# Autodesk Inventor assembly: pince
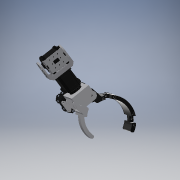
[picture p0: Inventor's stored thumbnail of the model, 180x180]
Saved by Autodesk Inventor 2017 (Build 210142000, 142)
## iProperties
Created: 2017-04-16
Part Number: pince
Document SubType Name: Assembly
Designer: franc
Author: franc
## Documents named in this file (8)
- C:\Users\franc\Desktop\EsialRobotik\Mecanique\robot-2017\pince\pince.iam
- C:\Users\franc\Desktop\EsialRobotik\Mecanique\robot-2017\pince\fixationPince.iam
- C:\Users\franc\Desktop\EsialRobotik\Mecanique\robot-2017\AX12-minerai\ax12_wheel.ipt
- C:\Users\franc\Desktop\EsialRobotik\Mecanique\robot-2017\AX12-minerai\ax12_box.ipt
- C:\Users\franc\Desktop\EsialRobotik\Mecanique\robot-2017\AX12-minerai\F2.ipt
- C:\Users\franc\Desktop\EsialRobotik\Mecanique\robot-2017\AX12-minerai\F3.ipt
- C:\Users\franc\Desktop\EsialRobotik\Mecanique\robot-2017\pince\pinceDroite.ipt
- C:\Users\franc\Desktop\EsialRobotik\Mecanique\robot-2017\pince\pinceGaucheMini.iam
## Components (11 placed, 7 different names)
1. fixationPince:1 [sub-assembly] — Mate:8, Mate:9, Mate:10, Mate:11, Mate:23, Mate:26, Mate:30, Mate:31, Mate:33, Mate:34
2. ax12_wheel:1 — Mate:29, Mate:32
3. ax12_box:1 — Mate:8, Mate:30, Mate:31, Mate:32
4. ax12_wheel:2 — Mate:9, Mate:10, Mate:11
5. ax12_box:2 — Mate:20, Mate:21, Mate:22
6. ax12_wheel:3
7. ax12_box:3 — Mate:17, Mate:18, Mate:19
8. F2:1 — Mate:20, Mate:21, Mate:22
9. F3:1 — Mate:17, Mate:18, Mate:19
10. pinceDroite:1 — Mate:23, Mate:26, Mate:29
11. pinceGaucheMini:1 [sub-assembly] — Mate:33, Mate:34
## Relationships (23: Mate 21, Insert 2)
- Mate:8: fixationPince:1 ↔ ax12_box:1
- [Insert]: ax12_wheel:2 ↔ ax12_box:2
- Mate:9: fixationPince:1 ↔ ax12_wheel:2
- Mate:10: fixationPince:1 ↔ ax12_wheel:2
- Mate:11: fixationPince:1 ↔ ax12_wheel:2
- [Insert]: ax12_wheel:3 ↔ ax12_box:3
- [Mate]: ax12_wheel:3 ↔ F2:1
- [Mate]: ax12_wheel:3 ↔ F2:1
- [Mate]: ax12_wheel:3 ↔ F2:1
- Mate:17: ax12_box:3 ↔ F3:1
- Mate:18: ax12_box:3 ↔ F3:1
- Mate:19: ax12_box:3 ↔ F3:1
- Mate:20: ax12_box:2 ↔ F2:1
- Mate:21: ax12_box:2 ↔ F2:1
- Mate:22: ax12_box:2 ↔ F2:1
- Mate:23: fixationPince:1 ↔ pinceDroite:1
- Mate:26: fixationPince:1 ↔ pinceDroite:1
- Mate:29: ax12_wheel:1 ↔ pinceDroite:1
- Mate:30: fixationPince:1 ↔ ax12_box:1
- Mate:31: fixationPince:1 ↔ ax12_box:1
- Mate:32: ax12_wheel:1 ↔ ax12_box:1
- Mate:33: fixationPince:1 ↔ pinceGaucheMini:1
- Mate:34: fixationPince:1 ↔ pinceGaucheMini:1
## Named parameters: d9_d1 = 0 mm, d16_d1 = 0 mm
